# Autodesk Inventor assembly: S901D
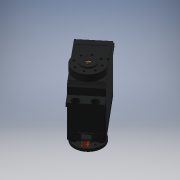
[picture p0: Inventor's stored thumbnail of the model, 180x180]
Saved by Autodesk Inventor 2016 (Build 200138000, 138)
## iProperties
Created: 2013-07-12
Part Number: S901D
Document SubType Name: Assembly
Designer: Maurice
Author: Maurice
## Documents named in this file (9)
- H:\CAD\Hexapod\turnigy-tgy-s901d-digital-servo-1.snapshot.5 (1)\S901D.iam
- H:\CAD\Hexapod\turnigy-tgy-s901d-digital-servo-1.snapshot.5 (1)\bottom-plate.ipt
- H:\CAD\Hexapod\turnigy-tgy-s901d-digital-servo-1.snapshot.5 (1)\housing.ipt
- H:\CAD\Hexapod\turnigy-tgy-s901d-digital-servo-1.snapshot.5 (1)\top-plate.ipt
- H:\CAD\Hexapod\turnigy-tgy-s901d-digital-servo-1.snapshot.5 (1)\pinion.ipt
- H:\CAD\Hexapod\turnigy-tgy-s901d-digital-servo-1.snapshot.5 (1)\top-arm.ipt
- H:\CAD\Hexapod\turnigy-tgy-s901d-digital-servo-1.snapshot.5 (1)\bottom-arm.ipt
- H:\CAD\Hexapod\turnigy-tgy-s901d-digital-servo-1.snapshot.5 (1)\long-screw.ipt
- H:\CAD\Hexapod\turnigy-tgy-s901d-digital-servo-1.snapshot.5 (1)\wire.ipt
## Components (11 placed, 8 different names)
1. bottom-plate:1 — Mate:1, Mate:2, Insert:1, Insert:2, Insert:3, Insert:4, Rotational:2, Insert:10, Insert:11, Insert:12, Insert:13, Mate:3, Mate:4, Mate:5
2. housing:1 — Insert:1, Insert:2, Insert:3, Insert:4, Insert:5, Insert:6, Insert:7, Insert:8
3. top-plate:1 — Insert:5, Insert:6, Insert:7, Insert:8, Rotational:1
4. pinion:1 — Rotational:1, Rigid:1
5. wire:1 — Mate:3, Mate:4, Mate:5
6. top-arm:1 — Rigid:1
7. bottom-arm:1 — Rotational:2
8. long-screw:1 — Insert:11
9. long-screw:2 — Insert:10
10. long-screw:3 — Insert:12
11. long-screw:4 — Insert:13
## Relationships (20: Insert 12, Mate 5, RevoluteJoint 2, WeldJoint 1)
- Mate:1: bottom-plate:1
- Mate:2: bottom-plate:1
- Insert:1: bottom-plate:1 ↔ housing:1
- Insert:2: bottom-plate:1 ↔ housing:1
- Insert:3: bottom-plate:1 ↔ housing:1
- Insert:4: bottom-plate:1 ↔ housing:1
- Insert:5: housing:1 ↔ top-plate:1
- Insert:6: housing:1 ↔ top-plate:1
- Insert:7: housing:1 ↔ top-plate:1
- Insert:8: housing:1 ↔ top-plate:1
- Rotational:1 [RevoluteJoint]: top-plate:1 ↔ pinion:1
- Rotational:2 [RevoluteJoint]: bottom-plate:1 ↔ bottom-arm:1
- Rigid:1 [WeldJoint]: pinion:1 ↔ top-arm:1
- Insert:10: bottom-plate:1 ↔ long-screw:2
- Insert:11: bottom-plate:1 ↔ long-screw:1
- Insert:12: bottom-plate:1 ↔ long-screw:3
- Insert:13: bottom-plate:1 ↔ long-screw:4
- Mate:3: bottom-plate:1 ↔ wire:1
- Mate:4: bottom-plate:1 ↔ wire:1
- Mate:5: bottom-plate:1 ↔ wire:1
